# Autodesk Inventor assembly: Assembly1
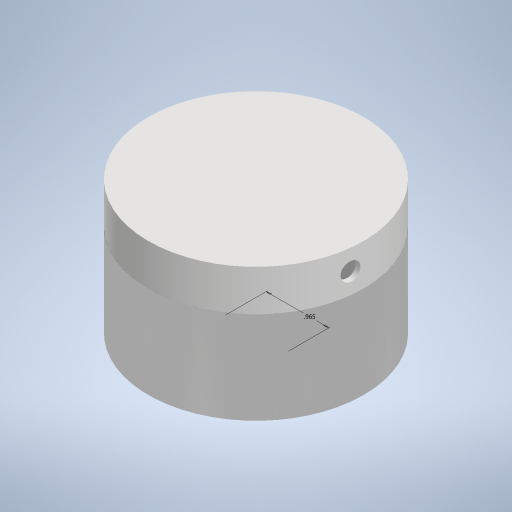
[picture p0: Inventor's stored thumbnail of the model, 512x512]
Saved by Autodesk Inventor 2023 (Build 270158000, 158)
## iProperties
Created: 2023-01-27
Part Number: Assembly1
Document SubType Name: Assembly
Designer: remidm
Author: remidm
## Documents named in this file (4)
- C:\Projects\Salt RPP\permeation_rig\design\InnerVessel.iam
- C:\Projects\Salt RPP\permeation_rig\design\DownstreamVolume.ipt
- C:\Projects\Salt RPP\permeation_rig\design\salt.ipt
- C:\Projects\Salt RPP\permeation_rig\design\UpstreamVolume.ipt
## Components (3 placed, 3 different names)
1. DownstreamVolume:1 — Mate:1, Mate:14, Mate:15, Mate:16, Mate:17, Mate:18
2. salt:1 — Mate:1, Mate:16
3. UpstreamVolume:1 — Mate:17, Mate:18
## Relationships (6: Mate 6)
- Mate:1: DownstreamVolume:1 ↔ salt:1
- Mate:14: DownstreamVolume:1
- Mate:15: DownstreamVolume:1
- Mate:16: DownstreamVolume:1 ↔ salt:1
- Mate:17: DownstreamVolume:1 ↔ UpstreamVolume:1
- Mate:18: DownstreamVolume:1 ↔ UpstreamVolume:1
